# Autodesk Inventor assembly: Button Fixture Assembly
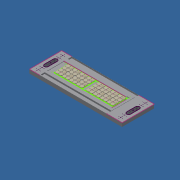
[picture p0: Inventor's stored thumbnail of the model, 180x180]
Saved by Autodesk Inventor 2016 (Build 200138000, 138)
## iProperties
Created: 2016-07-07
Part Number: Button Fixture Assembly
Document SubType Name: Assembly
Designer: Sam Clay
Author: Sam Clay
## Documents named in this file (3)
- Z:\enclosure\inventor\Button Fixture Assembly.iam
- Z:\enclosure\inventor\Button Fixture Base.ipt
- Z:\enclosure\inventor\Case Buttons CAM.ipt
## Components (17 placed, 2 different names)
1. Button Fixture Base:1 — Planar:2, Mate:1, Mate:2
2. Case Buttons CAM:1 — Planar:2, Mate:1, Mate:2
3. Case Buttons CAM:2
4. Case Buttons CAM:3
5. Case Buttons CAM:4
6. Case Buttons CAM:5
7. Case Buttons CAM:6
8. Case Buttons CAM:7
9. Case Buttons CAM:8
10. Case Buttons CAM:9
11. Case Buttons CAM:10
12. Case Buttons CAM:11
13. Case Buttons CAM:12
14. Case Buttons CAM:13
15. Case Buttons CAM:14
16. Case Buttons CAM:15
17. Case Buttons CAM:16
## Component patterns: (2 elements), (8 elements, first: Case Buttons CAM:1), Component Pattern 1:2 (8 elements)
## Relationships (3: Mate 2, PlanarJoint 1)
- Planar:2: Button Fixture Base:1 ↔ Case Buttons CAM:1
- Mate:1 (3.175 mm): Button Fixture Base:1 ↔ Case Buttons CAM:1
- Mate:2 (6.35 mm): Button Fixture Base:1 ↔ Case Buttons CAM:1
